# Autodesk Inventor assembly: Frame
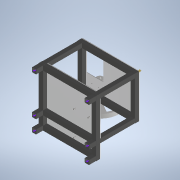
[picture p0: Inventor's stored thumbnail of the model, 180x180]
Saved by Autodesk Inventor 2022.2 (Build 262287000, 287)
## iProperties
_SolveAssemblyDoc: Frame Generator Solve Assembly
_Version: 25.0.0
Created: 2022-02-09
Part Number: Frame
Document SubType Name: Assembly
Designer: USUARIO
Author: USUARIO
## Documents named in this file (12)
- C:\Users\USUARIO\Downloads\Proyecto diseño\Frame.iam
- C:\Users\USUARIO\Downloads\Proyecto diseño\Pieza20.ipt
- C:\Users\USUARIO\Downloads\Proyecto diseño\Frame\Frame\Frame 1644558663413.iam
- C:\Users\USUARIO\Downloads\Proyecto diseño\Pieza26.ipt
- C:\Users\USUARIO\Downloads\Proyecto diseño\Carcasa.ipt
- C:\Users\USUARIO\Downloads\Proyecto diseño\Pieza35.ipt
- C:\Users\USUARIO\Downloads\Proyecto diseño\Shaft1.ipt
- C:\Users\USUARIO\Downloads\Proyecto diseño\Ensamble motor.iam
- C:\Users\USUARIO\Documents\Inventor\Content Center Files\R2022\es-ES\ANSI B18.2.1(3)\ANSI B18.2.1 - 7_16-14 UNC - 1,25(3).ipt
- C:\Users\USUARIO\Documents\Inventor\Content Center Files\R2022\es-ES\AS 1110\AS 1110 - M6 x 12.ipt
- C:\Users\USUARIO\Downloads\Proyecto diseño\Pieza43.ipt
- C:\Users\USUARIO\Downloads\Proyecto diseño\Pieza44.ipt
## Components (21 placed, 11 different names)
1. Pieza20:1 — Coincidencia:3
2. Frame 1644558663413:1 [sub-assembly] — Coincidencia:1, Nivelación:1, Nivelación:2, Coincidencia:4, Nivelación:3, Coincidencia:5, Coincidencia:9
3. Pieza26:1 — Coincidencia:1, Nivelación:1, Nivelación:2, Coincidencia:2, Coincidencia:3, Nivelación:4, Insertar:1
4. Carcasa:1 — Coincidencia:2, Coincidencia:6, Coincidencia:7, Nivelación:4, Insertar:1, Insertar:10, Insertar:11, Insertar:12, Insertar:13
5. Pieza35:1 — Coincidencia:4, Nivelación:3, Coincidencia:5, Coincidencia:8
6. Shaft:1 — Coincidencia:6, Coincidencia:7, Nivelación:5, Coincidencia:10, Nivelación:6
7. Ensamble motor:1 [sub-assembly] — Coincidencia:8, Nivelación:5, Coincidencia:9, Insertar:2, Insertar:3, Insertar:4, Insertar:5, Insertar:6, Insertar:7, Insertar:8, Insertar:9, Coincidencia:11, Nivelación:7
8. Tornillo de cabeza hex. - Pulgadas 7/16-14 UNC - 1,25:1 — Insertar:9
9. Tornillo de cabeza hex. - Pulgadas 7/16-14 UNC - 1,25:2 — Insertar:7
10. Tornillo de cabeza hex. - Pulgadas 7/16-14 UNC - 1,25:3 — Insertar:8
11. Tornillo de cabeza hex. - Pulgadas 7/16-14 UNC - 1,25:4 — Insertar:6
12. Tornillo de cabeza hex. - Pulgadas 7/16-14 UNC - 1,25:5 — Insertar:4
13. Tornillo de cabeza hex. - Pulgadas 7/16-14 UNC - 1,25:6 — Insertar:3
14. Tornillo de cabeza hex. - Pulgadas 7/16-14 UNC - 1,25:7 — Insertar:2
15. Tornillo de cabeza hex. - Pulgadas 7/16-14 UNC - 1,25:8 — Insertar:5
16. AS 1110 - Métrico M6 x 12:1 — Insertar:12
17. AS 1110 - Métrico M6 x 12:2 — Insertar:10
18. AS 1110 - Métrico M6 x 12:3 — Insertar:11
19. AS 1110 - Métrico M6 x 12:4 — Insertar:13
20. Pieza43:1 — Coincidencia:10, Nivelación:6
21. Pieza44:1 — Coincidencia:11, Nivelación:7
## Relationships (31: Insert 13, Mate 11, Flush 7)
- Coincidencia:1 [Mate]: Frame 1644558663413:1 ↔ Pieza26:1
- Nivelación:1 [Flush]: Frame 1644558663413:1 ↔ Pieza26:1
- Nivelación:2 [Flush]: Frame 1644558663413:1 ↔ Pieza26:1
- Coincidencia:2 [Mate]: Pieza26:1 ↔ Carcasa:1
- Coincidencia:3 [Mate]: Pieza20:1 ↔ Pieza26:1
- Coincidencia:4 [Mate]: Frame 1644558663413:1 ↔ Pieza35:1
- Nivelación:3 [Flush]: Frame 1644558663413:1 ↔ Pieza35:1
- Coincidencia:5 [Mate]: Frame 1644558663413:1 ↔ Pieza35:1
- Coincidencia:6 [Mate]: Carcasa:1 ↔ Shaft:1
- Coincidencia:7 [Mate] (1 mm): Carcasa:1 ↔ Shaft:1
- Nivelación:4 [Flush]: Pieza26:1 ↔ Carcasa:1
- Coincidencia:8 [Mate]: Pieza35:1 ↔ Ensamble motor:1
- Nivelación:5 [Flush]: Shaft:1 ↔ Ensamble motor:1
- Coincidencia:9 [Mate] (4.966 mm): Frame 1644558663413:1 ↔ Ensamble motor:1
- Insertar:1: Pieza26:1 ↔ Carcasa:1
- Insertar:2: Ensamble motor:1 ↔ Tornillo de cabeza hex. - Pulgadas 7/16-14 UNC - 1,25:7
- Insertar:3: Ensamble motor:1 ↔ Tornillo de cabeza hex. - Pulgadas 7/16-14 UNC - 1,25:6
- Insertar:4: Ensamble motor:1 ↔ Tornillo de cabeza hex. - Pulgadas 7/16-14 UNC - 1,25:5
- Insertar:5: Ensamble motor:1 ↔ Tornillo de cabeza hex. - Pulgadas 7/16-14 UNC - 1,25:8
- Insertar:6: Ensamble motor:1 ↔ Tornillo de cabeza hex. - Pulgadas 7/16-14 UNC - 1,25:4
- Insertar:7: Ensamble motor:1 ↔ Tornillo de cabeza hex. - Pulgadas 7/16-14 UNC - 1,25:2
- Insertar:8: Ensamble motor:1 ↔ Tornillo de cabeza hex. - Pulgadas 7/16-14 UNC - 1,25:3
- Insertar:9: Ensamble motor:1 ↔ Tornillo de cabeza hex. - Pulgadas 7/16-14 UNC - 1,25:1
- Insertar:10: Carcasa:1 ↔ AS 1110 - Métrico M6 x 12:2
- Insertar:11: Carcasa:1 ↔ AS 1110 - Métrico M6 x 12:3
- Insertar:12: Carcasa:1 ↔ AS 1110 - Métrico M6 x 12:1
- Insertar:13: Carcasa:1 ↔ AS 1110 - Métrico M6 x 12:4
- Coincidencia:10 [Mate]: Shaft:1 ↔ Pieza43:1
- Nivelación:6 [Flush]: Shaft:1 ↔ Pieza43:1
- Coincidencia:11 [Mate]: Ensamble motor:1 ↔ Pieza44:1
- Nivelación:7 [Flush]: Ensamble motor:1 ↔ Pieza44:1
